# Autodesk Inventor assembly: Cooper3.0
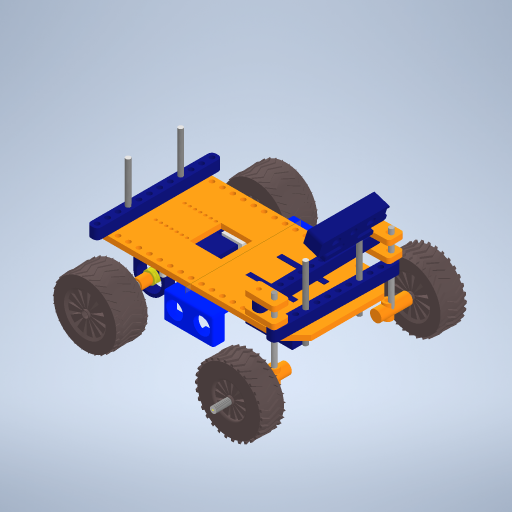
[picture p0: Inventor's stored thumbnail of the model, 512x512]
Saved by Autodesk Inventor 2024.3 (Build 283343000, 343)
## iProperties
Created: 2024-03-25
Part Number: Cooper3.0
Document SubType Name: Assembly
Designer: JDAM
Author: JDAM
## Documents named in this file (36)
- C:\Users\JDAM\Documents\Modelos - inventor\Partes cooper\Cooper3.0.iam
- C:\Users\JDAM\Documents\Modelos - inventor\Partes cooper\dirección\soporte de direccion.ipt
- C:\Users\JDAM\Documents\Modelos - inventor\Partes cooper\Barra roscada4mm.ipt
- C:\Users\JDAM\Documents\Modelos - inventor\Partes cooper\Barra roscada4mm_MIR.ipt
- C:\Users\JDAM\Documents\Modelos - inventor\Partes cooper\dirección\codo_MIR.ipt
- C:\Users\JDAM\Documents\Modelos - inventor\Partes cooper\Chasis1.ipt
- C:\Users\JDAM\Documents\Modelos - inventor\Partes cooper\Barra roscada6mm.ipt
- C:\Users\JDAM\Documents\Modelos - inventor\Partes cooper\ruedasRefD.ipt
- C:\Users\JDAM\Documents\Modelos - inventor\Partes cooper\Piso volado\nano.ipt
- C:\Users\JDAM\Documents\Modelos - inventor\Partes cooper\ruedasRefT.ipt
- C:\Users\JDAM\Documents\Modelos - inventor\Partes cooper\Barra roscada4mm_MIR1.ipt
- C:\Users\JDAM\Documents\Modelos - inventor\Partes cooper\Barra roscada4mm_MIR2.ipt
- C:\Users\JDAM\Documents\Modelos - inventor\Partes cooper\Barra roscada4mm_MIR1_MIR.ipt
- C:\Users\JDAM\Documents\Modelos - inventor\Partes cooper\Chasis2.ipt
- C:\Users\JDAM\Documents\Modelos - inventor\Partes cooper\Piso volado\base del motor2.ipt
- C:\Users\JDAM\Documents\Modelos - inventor\Partes cooper\dirección\soporte de direccion_MIR.ipt
- C:\Users\JDAM\Downloads\ball_bearing_inner_race\ball_bearing_inner_race.ipt
- C:\Users\JDAM\Downloads\ball_bearing_inner_race\ball_bearing_inner_race_MIR.ipt
- C:\Users\JDAM\Documents\Modelos - inventor\Partes cooper\Piso volado\acople.ipt
- C:\Users\JDAM\Documents\Modelos - inventor\Partes cooper\Piso volado\acople2.ipt
- C:\Users\JDAM\Documents\Modelos - inventor\Partes cooper\Piso volado\acople_MIR.ipt
- C:\Users\JDAM\Documents\Modelos - inventor\Partes cooper\Piso volado\acople2_MIR.ipt
- C:\Users\JDAM\Documents\Modelos - inventor\Partes cooper\Barra roscada6mm_MIR2.ipt
- C:\Users\JDAM\Documents\Modelos - inventor\Partes cooper\ruedasRefT_MIR1.ipt
- C:\Users\JDAM\Documents\Modelos - inventor\Partes cooper\dirección\codo_MIR_MIR.ipt
- C:\Users\JDAM\Documents\Modelos - inventor\Partes cooper\Barra roscada6mm_MIR3.ipt
- C:\Users\JDAM\Documents\Modelos - inventor\Partes cooper\ruedasRefD_MIR1.ipt
- C:\Users\JDAM\Documents\Modelos - inventor\Partes cooper\dirección\angulo.ipt
- C:\Users\JDAM\Documents\Modelos - inventor\Partes cooper\dirección\angulo_MIR.ipt
- C:\Users\JDAM\Documents\Modelos - inventor\Partes cooper\dirección\soporte de direccion2.ipt
- C:\Users\JDAM\Documents\Modelos - inventor\Partes cooper\dirección\angulo_MIR1.ipt
- C:\Users\JDAM\Documents\Modelos - inventor\Partes cooper\camara-soporte\soporte-azul.ipt
- C:\Users\JDAM\Documents\Modelos - inventor\Partes cooper\camara-soporte\ultra.ipt
- C:\Users\JDAM\Documents\Modelos - inventor\Partes cooper\camara-soporte\ultra_MIR.ipt
- C:\Users\JDAM\Documents\Modelos - inventor\Partes cooper\camara-soporte\ultra_MIR1.ipt
- C:\Users\JDAM\Documents\Modelos - inventor\Partes cooper\Piso volado\base del motor3t.ipt
## Components (39 placed, 35 different names)
1. soporte de direccion:1 — Rotational:2, Rotational:3, Rotational:10, Rotational:11
2. Barra roscada4mm:2 — Rotational:11
3. Barra roscada4mm_MIR:1 — Rotational:10, Rotational:12, Rotational:13
4. codo_MIR:1 — Rigid:2
5. Chasis1:1 — Rotational:2, Flush:1, Mate:4, Mate:5, Rotational:5, Rotational:15
6. Barra roscada6mm:1 — Rigid:2, Rigid:3
7. ruedasRefD:1 — Rigid:3
8. nano:1 — Mate:4, Mate:5
9. ruedasRefT:1 — Rotational:9
10. Barra roscada4mm:3 — Rotational:3, Rotational:4
11. Barra roscada4mm_MIR1:1
12. Barra roscada4mm_MIR2:1
13. Barra roscada4mm_MIR1_MIR:1
14. Chasis2:1 — Rotational:4
15. base del motor2:1 — Rotational:5, Mate:6
16. soporte de direccion_MIR:1
17. ball_bearing_inner_race:1 — Mate:6
18. ball_bearing_inner_race_MIR:1 — Rotational:6
19. acople:1 — Rotational:6, Rotational:7
20. acople2:1 — Rotational:7
21. acople_MIR:1 — Rotational:8
22. acople2_MIR:1 — Rotational:8, Rigid:5
23. Barra roscada6mm:2 — Rigid:5
24. Barra roscada6mm_MIR2:1 — Rotational:9
25. ruedasRefT_MIR1:1
26. codo_MIR_MIR:1 — Rigid:6
27. Barra roscada6mm_MIR3:1 — Rigid:6, Rigid:7
28. ruedasRefD_MIR1:1 — Rigid:7
29. angulo:1 — Rotational:12
30. angulo:2 — Rotational:13
31. angulo_MIR:1 — Rotational:14
32. soporte de direccion2:1 — Rotational:14
33. angulo_MIR1:1
34. soporte-azul:1
35. ultra:1 — Rotational:15
36. ultra_MIR:1
37. ultra:2
38. ultra_MIR1:1
39. base del motor3t:1
## Relationships (23: RevoluteJoint 14, WeldJoint 5, Mate 3, Flush 1)
- Rotational:2 [RevoluteJoint] (10 mm): soporte de direccion:1 ↔ Chasis1:1
- Rigid:2 [WeldJoint]: codo_MIR:1 ↔ Barra roscada6mm:1
- Rigid:3 [WeldJoint] (-15 mm): Barra roscada6mm:1 ↔ ruedasRefD:1
- Flush:1 (-100 mm): Chasis1:1
- Rotational:3 [RevoluteJoint] (30 mm): soporte de direccion:1 ↔ Barra roscada4mm:3
- Rotational:4 [RevoluteJoint]: Barra roscada4mm:3 ↔ Chasis2:1
- Mate:4: Chasis1:1 ↔ nano:1
- Mate:5: Chasis1:1 ↔ nano:1
- Rotational:5 [RevoluteJoint]: Chasis1:1 ↔ base del motor2:1
- Mate:6: base del motor2:1 ↔ ball_bearing_inner_race:1
- Rotational:6 [RevoluteJoint] (10 mm): ball_bearing_inner_race_MIR:1 ↔ acople:1
- Rotational:7 [RevoluteJoint] (7 mm): acople:1 ↔ acople2:1
- Rotational:8 [RevoluteJoint] (-7 mm): acople_MIR:1 ↔ acople2_MIR:1
- Rigid:5 [WeldJoint]: acople2_MIR:1 ↔ Barra roscada6mm:2
- Rotational:9 [RevoluteJoint] (-20 mm): ruedasRefT:1 ↔ Barra roscada6mm_MIR2:1
- Rotational:10 [RevoluteJoint] (-28 mm): soporte de direccion:1 ↔ Barra roscada4mm_MIR:1
- Rotational:11 [RevoluteJoint] (-28 mm): soporte de direccion:1 ↔ Barra roscada4mm:2
- Rigid:6 [WeldJoint]: codo_MIR_MIR:1 ↔ Barra roscada6mm_MIR3:1
- Rigid:7 [WeldJoint] (-15 mm): Barra roscada6mm_MIR3:1 ↔ ruedasRefD_MIR1:1
- Rotational:12 [RevoluteJoint] (-10 mm): Barra roscada4mm_MIR:1 ↔ angulo:1
- Rotational:13 [RevoluteJoint] (20 mm): Barra roscada4mm_MIR:1 ↔ angulo:2
- Rotational:14 [RevoluteJoint]: angulo_MIR:1 ↔ soporte de direccion2:1
- Rotational:15 [RevoluteJoint]: Chasis1:1 ↔ ultra:1
